# Autodesk Inventor assembly: DrivetrainSupport
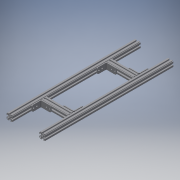
[picture p0: Inventor's stored thumbnail of the model, 180x180]
Saved by Autodesk Inventor 2018 (Build 220112000, 112)
## iProperties
Created: 2018-08-26
Part Number: DrivetrainSupport
Document SubType Name: Assembly
Designer: anirudh
Author: anirudh
## Documents named in this file (4)
- C:\Users\anirudh\Documents\MARS Fund\Silicon Edge\2018-2019\DrivetrainSupport.iam
- C:\Users\anirudh\Documents\MARS Fund\Silicon Edge\2018-2019\12.6inREV.ipt
- C:\Users\anirudh\Documents\MARS Fund\Silicon Edge\2018-2019\67mmREV.ipt
- C:\Users\anirudh\Documents\MARS Fund\Silicon Edge\2018-2019\LBracket.ipt
## Components (8 placed, 3 different names)
1. 12.6inREV:1 — Angle:1, Angle:2, Flush:1, Flush:2, Mate:1, Flush:3, Flush:4, Mate:2, Flush:6, Flush:7, Mate:5, Flush:8, Mate:7, Flush:9, Flush:10
2. 12.6inREV:2 — Flush:5, Flush:6, Mate:3, Mate:9, Mate:11
3. 67mmREV:1 — Angle:1, Flush:1, Flush:2, Mate:1, Flush:5, Mate:3, Mate:4, Mate:8
4. 67mmREV:2 — Angle:2, Flush:3, Flush:4, Mate:2, Mate:6, Mate:10
5. LBracket:1 — Flush:7, Mate:4, Mate:5
6. LBracket:2 — Flush:8, Mate:6, Mate:7
7. LBracket:3 — Flush:9, Mate:8, Mate:9
8. LBracket:4 — Flush:10, Mate:10, Mate:11
## Relationships (23: Mate 11, Flush 10, Angle 2)
- Angle:1 (90 deg): 12.6inREV:1 ↔ 67mmREV:1
- Angle:2 (90 deg): 12.6inREV:1 ↔ 67mmREV:2
- Flush:1: 12.6inREV:1 ↔ 67mmREV:1
- Flush:2 (-70.815 mm): 12.6inREV:1 ↔ 67mmREV:1
- Mate:1: 12.6inREV:1 ↔ 67mmREV:1
- Flush:3 (70.815 mm): 12.6inREV:1 ↔ 67mmREV:2
- Flush:4: 12.6inREV:1 ↔ 67mmREV:2
- Mate:2: 12.6inREV:1 ↔ 67mmREV:2
- Flush:5: 12.6inREV:2 ↔ 67mmREV:1
- Flush:6: 12.6inREV:1 ↔ 12.6inREV:2
- Mate:3: 12.6inREV:2 ↔ 67mmREV:1
- Flush:7: 12.6inREV:1 ↔ LBracket:1
- Mate:4: 67mmREV:1 ↔ LBracket:1
- Mate:5: 12.6inREV:1 ↔ LBracket:1
- Flush:8: 12.6inREV:1 ↔ LBracket:2
- Mate:6: 67mmREV:2 ↔ LBracket:2
- Mate:7: 12.6inREV:1 ↔ LBracket:2
- Flush:9: 12.6inREV:1 ↔ LBracket:3
- Mate:8: 67mmREV:1 ↔ LBracket:3
- Mate:9: 12.6inREV:2 ↔ LBracket:3
- Flush:10: 12.6inREV:1 ↔ LBracket:4
- Mate:10: 67mmREV:2 ↔ LBracket:4
- Mate:11: 12.6inREV:2 ↔ LBracket:4
